# Autodesk Inventor assembly: FinalAssembly_1
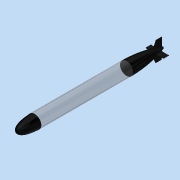
[picture p0: Inventor's stored thumbnail of the model, 180x180]
Saved by Autodesk Inventor 2017 (Build 210142000, 142)
## iProperties
Created: 2016-09-09
Part Number: FinalAssembly_1
Document SubType Name: Assembly
Designer: techn
Author: techn
## Documents named in this file (5)
- D:\OneDrive\Documents\Other Projects\Submarine\CAD\FinalAssembly_1.iam
- D:\OneDrive\Documents\Other Projects\Submarine\CAD\midships\PrimaryHullLexanTube_01.ipt
- D:\OneDrive\Documents\Other Projects\Submarine\CAD\fore\primarySingleFore_02.ipt
- D:\OneDrive\Documents\Other Projects\Submarine\CAD\aft\PrimarySingleAft_03.ipt
- D:\OneDrive\Documents\Other Projects\Submarine\CAD\aft\RearmostAftSectionAssembly0.iam
## Components (4 placed, 4 different names)
1. PrimaryHullLexanTube_01:1 — Mate:1, Mate:2, Mate:3, Mate:4, Tangent:1
2. primarySingleFore_02:1 — Mate:3, Mate:4
3. PrimarySingleAft_03:1 — Mate:1, Mate:2, Mate:5, Flush:2
4. RearmostAftSectionAssembly0:1 [sub-assembly] — Mate:5, Flush:2
## Relationships (9: Mate 5, Flush 2, Angle 1, Tangent 1)
- Mate:1: PrimaryHullLexanTube_01:1 ↔ PrimarySingleAft_03:1
- Mate:2: PrimaryHullLexanTube_01:1 ↔ PrimarySingleAft_03:1
- Mate:3: PrimaryHullLexanTube_01:1 ↔ primarySingleFore_02:1
- Mate:4: PrimaryHullLexanTube_01:1 ↔ primarySingleFore_02:1
- Angle:1 (0 deg)
- Tangent:1: PrimaryHullLexanTube_01:1
- Flush:1 (-50.8 mm)
- Mate:5: PrimarySingleAft_03:1 ↔ RearmostAftSectionAssembly0:1
- Flush:2: PrimarySingleAft_03:1 ↔ RearmostAftSectionAssembly0:1
